# Autodesk Inventor assembly: ArmDriver
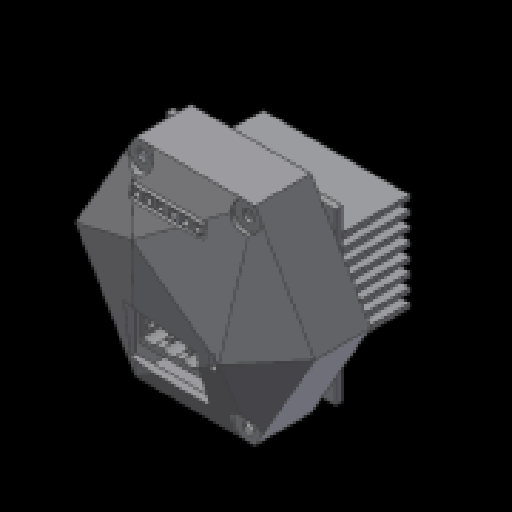
[picture p0: Inventor's stored thumbnail of the model, 512x512]
Saved by Autodesk Inventor 2025.2 (Build 292293000, 293)
## iProperties
Created: 2023-12-09
Part Number: ArmDriver
Document SubType Name: Assembly
Designer: valer
Author: valer
## Documents named in this file (3)
- C:\Users\valer\Desktop\str1ker\cad\ArmDriver.iam
- C:\Users\valer\Desktop\str1ker\cad\external\ArmDriver\IBTMini.ipt
- C:\Users\valer\Desktop\str1ker\cad\ArmDriverBoardCover.ipt
## Components (2 placed, 2 different names)
1. IBTMini:1 — Flush:1
2. ArmDriverBoardCover:1 — Flush:1
## Relationships (1: Flush 1)
- Flush:1: IBTMini:1 ↔ ArmDriverBoardCover:1
